# Autodesk Inventor assembly: YCart
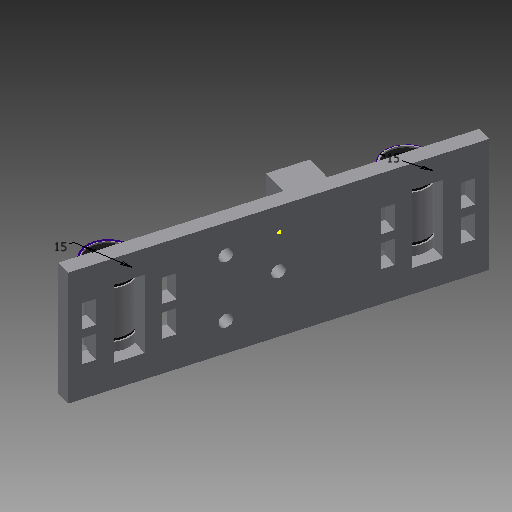
[picture p0: Inventor's stored thumbnail of the model, 512x512]
Saved by Autodesk Inventor 2019 (Build 230136000, 136)
## iProperties
Created: 2019-08-21
Part Number: YCart
Document SubType Name: Assembly
Designer: Bruno
Author: Bruno
## Documents named in this file (4)
- C:\Users\Bruno\Stuff\Ajedrez2\YCart.iam
- C:\Users\Bruno\Stuff\Ajedrez2\YCartFloor.ipt
- C:\Users\Bruno\Stuff\Ajedrez2\Lm8uu.ipt
- C:\Users\Bruno\Stuff\Ajedrez\Inkjet Printer Prototype\Workspace\YCartBeltClamp.ipt
## Components (4 placed, 3 different names)
1. YCartFloor:1 — Rigid:1, Rigid:2, Flush:1
2. Lm8uu:1 — Rigid:1
3. Lm8uu:2 — Rigid:2
4. YCartBeltClamp:1 — Flush:1
## Relationships (3: WeldJoint 2, Flush 1)
- Rigid:1 [WeldJoint]: YCartFloor:1 ↔ Lm8uu:1
- Rigid:2 [WeldJoint]: YCartFloor:1 ↔ Lm8uu:2
- Flush:1: YCartFloor:1 ↔ YCartBeltClamp:1
